# Autodesk Inventor assembly: Assieme 1 - Trasporto
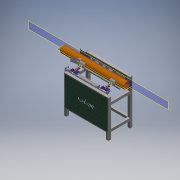
[picture p0: Inventor's stored thumbnail of the model, 180x180]
Saved by Autodesk Inventor 2018 (Build 220112000, 112)
## iProperties
Created: 2020-05-30
Part Number: Assieme 1 - Trasporto
Material: Generico
Document SubType Name: Weldment
Designer: Francesco
Weld Material: Welded Aluminum-6061
Author: Francesco
## Documents named in this file (12)
- C:\Users\Francesco\no-brim\Meccanica\Progetto Inventor no-brim\Assiemi\Assieme 1 - Trasporto.iam
- C:\Users\Francesco\no-brim\Meccanica\Progetto Inventor no-brim\Assiemi\Telaio - Trasporto.iam
- C:\Users\Francesco\no-brim\Meccanica\Progetto Inventor no-brim\Assiemi\Rulliera - Trasporto.iam
- C:\Users\Francesco\no-brim\Meccanica\Progetto Inventor no-brim\Parti\Lamiera riferimento.ipt
- C:\Users\Francesco\no-brim\Meccanica\Progetto Inventor no-brim\Parti\Spessore plastica.ipt
- C:\Users\Francesco\no-brim\Meccanica\Progetto Inventor no-brim\Parti\Tubo.ipt
- C:\Users\Francesco\no-brim\Meccanica\Progetto Inventor no-brim\Assiemi\Pistoni pinza - Trasporto.iam
- C:\Users\Francesco\no-brim\Meccanica\Progetto Inventor no-brim\Parti\Asse lineare corsa 300 mm\Assieme asse lineare corsa 300 mm.iam
- C:\Users\Francesco\no-brim\Meccanica\Progetto Inventor no-brim\Parti\Lamiera logo no-brim.ipt
- C:\Users\Francesco\no-brim\Meccanica\Progetto Inventor no-brim\Assiemi\Supporto saldato pistone 2 - Trasporto.iam
- C:\Users\Francesco\no-brim\Meccanica\Progetto Inventor no-brim\Parti\Lamiera 10mm supporto asse.ipt
- C:\Users\Francesco\no-brim\Meccanica\Progetto Inventor no-brim\Parti\Lamiera ingresso tubo.ipt
## Components (16 placed, 11 different names)
1. Telaio - Trasporto:1 [sub-assembly] — Coincidente:1, Coincidente:2, Coincidente:3, Coincidente:4, Coincidente:5, Coincidente:6, Coincidente:7, Coincidente:8, Coincidente:9, Coincidente:10, Coincidente:11, Angolo:1, Angolo:3, Coincidente:16, Angolo:4, Coincidente:23, Allineato:14, Allineato:15, Coincidente:24, Coincidente:28, Allineato:19, Coincidente:32, Coincidente:33, Allineato:20
2. Rulliera - Trasporto:1 [sub-assembly] — Coincidente:1, Coincidente:5
3. Rulliera - Trasporto:2 [sub-assembly] — Coincidente:3, Coincidente:8
4. Rulliera - Trasporto:3 [sub-assembly] — Coincidente:2, Coincidente:6, Allineato:1
5. Rulliera - Trasporto:4 [sub-assembly] — Coincidente:4, Coincidente:7
6. Lamiera riferimento:1 — Coincidente:9, Coincidente:10, Coincidente:11, Coincidente:12, Coincidente:13, Coincidente:14, Coincidente:34
7. Spessore plastica:1 — Coincidente:12, Coincidente:13, Coincidente:14, Allineato:5
8. Tubo:1 — Angolo:1, Allineato:2, Angolo:2, Tangente:1, Coincidente:17
9. Pistoni pinza - Trasporto:1 [sub-assembly] — Angolo:3, Coincidente:16, Coincidente:17, Allineato:3, Allineato:4, Coincidente:19, Allineato:8, Allineato:9
10. Pistoni pinza - Trasporto:2 [sub-assembly] — Allineato:3, Allineato:4, Allineato:5, Coincidente:25, Coincidente:26
11. Assieme asse lineare corsa 300 mm:1 [sub-assembly] — Angolo:4, Coincidente:19, Allineato:7, Allineato:9, Coincidente:29, Coincidente:30, Coincidente:31
12. Lamiera logo no-brim:1 — Coincidente:23, Allineato:14, Allineato:15
13. Supporto saldato pistone 2:1 [sub-assembly] — Coincidente:24, Coincidente:25, Coincidente:26
14. Lamiera 10mm supporto asse:1 — Coincidente:28, Coincidente:29, Coincidente:30, Allineato:17, Allineato:18, Allineato:19
15. Lamiera 10mm supporto asse:2 — Allineato:17, Allineato:18, Coincidente:31
16. Lamiera ingresso:1 — Coincidente:32, Coincidente:33, Allineato:20
## Relationships (47: Mate 28, Flush 14, Angle 4, Tangent 1)
- Coincidente:1 [Mate]: Telaio - Trasporto:1 ↔ Rulliera - Trasporto:1
- Coincidente:2 [Mate]: Telaio - Trasporto:1 ↔ Rulliera - Trasporto:3
- Coincidente:3 [Mate]: Telaio - Trasporto:1 ↔ Rulliera - Trasporto:2
- Coincidente:4 [Mate]: Telaio - Trasporto:1 ↔ Rulliera - Trasporto:4
- Coincidente:5 [Mate]: Telaio - Trasporto:1 ↔ Rulliera - Trasporto:1
- Coincidente:6 [Mate]: Telaio - Trasporto:1 ↔ Rulliera - Trasporto:3
- Coincidente:7 [Mate]: Telaio - Trasporto:1 ↔ Rulliera - Trasporto:4
- Coincidente:8 [Mate]: Telaio - Trasporto:1 ↔ Rulliera - Trasporto:2
- Coincidente:9 [Mate]: Telaio - Trasporto:1 ↔ Lamiera riferimento:1
- Coincidente:10 [Mate]: Telaio - Trasporto:1 ↔ Lamiera riferimento:1
- Coincidente:11 [Mate] (5 mm): Telaio - Trasporto:1 ↔ Lamiera riferimento:1
- Coincidente:12 [Mate]: Lamiera riferimento:1 ↔ Spessore plastica:1
- Coincidente:13 [Mate]: Lamiera riferimento:1 ↔ Spessore plastica:1
- Coincidente:14 [Mate]: Lamiera riferimento:1 ↔ Spessore plastica:1
- Angolo:1 [Angle] (0 deg): Telaio - Trasporto:1 ↔ Tubo:1
- Allineato:1 [Flush] (13.5 mm): Rulliera - Trasporto:3
- Allineato:2 [Flush]: Tubo:1
- Angolo:2 [Angle] (0 deg): Tubo:1
- Tangente:1: Tubo:1
- Angolo:3 [Angle] (0 deg): Telaio - Trasporto:1 ↔ Pistoni pinza - Trasporto:1
- Coincidente:16 [Mate] (22 mm): Telaio - Trasporto:1 ↔ Pistoni pinza - Trasporto:1
- Coincidente:17 [Mate]: Tubo:1 ↔ Pistoni pinza - Trasporto:1
- Allineato:3 [Flush]: Pistoni pinza - Trasporto:1 ↔ Pistoni pinza - Trasporto:2
- Allineato:4 [Flush]: Pistoni pinza - Trasporto:1 ↔ Pistoni pinza - Trasporto:2
- Allineato:5 [Flush]: Spessore plastica:1 ↔ Pistoni pinza - Trasporto:2
- Angolo:4 [Angle] (0 deg): Telaio - Trasporto:1 ↔ Assieme asse lineare corsa 300 mm:1
- Coincidente:19 [Mate] (8 mm): Pistoni pinza - Trasporto:1 ↔ Assieme asse lineare corsa 300 mm:1
- Allineato:7 [Flush] (-55 mm): Assieme asse lineare corsa 300 mm:1
- Allineato:8 [Flush]: Pistoni pinza - Trasporto:1
- Allineato:9 [Flush]: Pistoni pinza - Trasporto:1 ↔ Assieme asse lineare corsa 300 mm:1
- Coincidente:23 [Mate]: Telaio - Trasporto:1 ↔ Lamiera logo no-brim:1
- Allineato:14 [Flush] (17.5 mm): Telaio - Trasporto:1 ↔ Lamiera logo no-brim:1
- Allineato:15 [Flush] (17.5 mm): Telaio - Trasporto:1 ↔ Lamiera logo no-brim:1
- Coincidente:24 [Mate]: Telaio - Trasporto:1 ↔ Supporto saldato pistone 2:1
- Coincidente:25 [Mate]: Pistoni pinza - Trasporto:2 ↔ Supporto saldato pistone 2:1
- Coincidente:26 [Mate]: Pistoni pinza - Trasporto:2 ↔ Supporto saldato pistone 2:1
- Coincidente:28 [Mate]: Telaio - Trasporto:1 ↔ Lamiera 10mm supporto asse:1
- Coincidente:29 [Mate]: Assieme asse lineare corsa 300 mm:1 ↔ Lamiera 10mm supporto asse:1
- Coincidente:30 [Mate] (30 mm): Assieme asse lineare corsa 300 mm:1 ↔ Lamiera 10mm supporto asse:1
- Allineato:17 [Flush]: Lamiera 10mm supporto asse:1 ↔ Lamiera 10mm supporto asse:2
- Allineato:18 [Flush]: Lamiera 10mm supporto asse:1 ↔ Lamiera 10mm supporto asse:2
- Coincidente:31 [Mate] (30 mm): Assieme asse lineare corsa 300 mm:1 ↔ Lamiera 10mm supporto asse:2
- Allineato:19 [Flush] (60 mm): Telaio - Trasporto:1 ↔ Lamiera 10mm supporto asse:1
- Coincidente:32 [Mate]: Telaio - Trasporto:1 ↔ Lamiera ingresso:1
- Coincidente:33 [Mate]: Telaio - Trasporto:1 ↔ Lamiera ingresso:1
- Allineato:20 [Flush]: Telaio - Trasporto:1 ↔ Lamiera ingresso:1
- Coincidente:34 [Mate]: Lamiera riferimento:1
